# Autodesk Inventor assembly: Assembly1
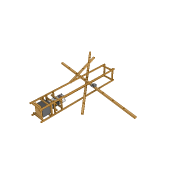
[picture p0: Inventor's stored thumbnail of the model, 180x180]
Saved by Autodesk Inventor 2020 (Build 240168000, 168)
## iProperties
Created: 2022-05-05
Part Number: Assembly1
Document SubType Name: Assembly
Designer: leo
Author: leo
## Documents named in this file (7)
- C:\Users\leo.DESKTOP-592E5E6\Documents\GitHub\TallerDix2022\cad\Inventor\Assembly1.iam
- C:\Users\leo.DESKTOP-592E5E6\Documents\GitHub\TallerDix2022\cad\Inventor\Base listones.ipt
- C:\Users\leo.DESKTOP-592E5E6\Documents\GitHub\TallerDix2022\cad\Inventor\adocreto.ipt
- C:\Users\leo.DESKTOP-592E5E6\Documents\GitHub\TallerDix2022\cad\Inventor\Caja motriz BASE.iam
- C:\Users\leo.DESKTOP-592E5E6\Documents\GitHub\TallerDix2022\cad\Inventor\pieza.ipt
- C:\Users\leo.DESKTOP-592E5E6\Documents\GitHub\TallerDix2022\cad\Inventor\parte móvil.iam
- C:\Users\leo.DESKTOP-592E5E6\Documents\GitHub\TallerDix2022\cad\Inventor\pieza2.ipt
## Components (6 placed, 6 different names)
1. Base listones:1
2. adocreto:1 — Flush:1, Flush:2
3. Caja motriz BASE:1 [sub-assembly] — Flush:3, Mate:4
4. parte móvil:1 [sub-assembly] — Mate:2, Mate:3, Mate:4, Insert:1
5. pieza:1 — Mate:5, Mate:6, Insert:2
6. pieza2:1 — Insert:1, Insert:2
## Relationships (10: Mate 5, Flush 3, Insert 2)
- Flush:1: adocreto:1
- Flush:2: adocreto:1
- Flush:3: Caja motriz BASE:1
- Mate:2 (1300 mm): parte móvil:1
- Mate:3 (200 mm): parte móvil:1
- Mate:4: Caja motriz BASE:1 ↔ parte móvil:1
- Mate:5 (-200 mm): pieza:1
- Mate:6 (1500 mm): pieza:1
- Insert:1 (10 mm): parte móvil:1 ↔ pieza2:1
- Insert:2: pieza:1 ↔ pieza2:1
